# Autodesk Inventor assembly: 足首_独立ピッチ_1
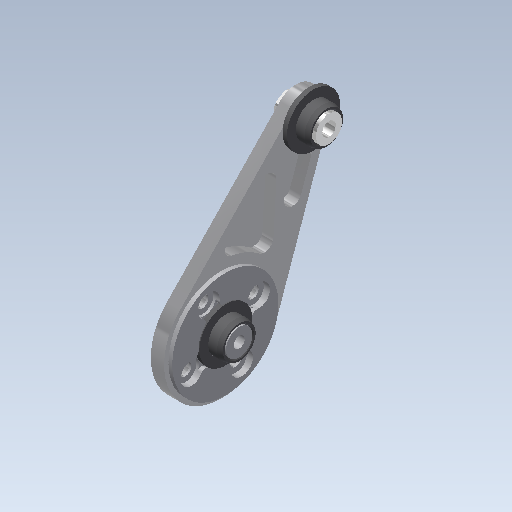
[picture p0: Inventor's stored thumbnail of the model, 512x512]
Saved by Autodesk Inventor 2020 (Build 240168000, 168)
## iProperties
Created: 2016-05-04
Part Number: 足首_独立ピッチ_1
Document SubType Name: Assembly
Designer: hiroaki
Mass: 12.4515 g
Surface Area: 78.9605 cm^2
Volume: 4.53639 cm^3
Density: 2.74481 g/cm^3
Author: hiroaki
## Documents named in this file (6)
- C:\Users\Masato\Desktop\最新版\OpenPlatform_ver3_0\下半身\足首\足首_独立ピッチ_1.iam
- C:\Users\Masato\Desktop\最新版\OpenPlatform_ver3_0\下半身\足首\足首_独立ピッチ_1_1.ipt
- C:\Users\Masato\Desktop\最新版\OpenPlatform_ver3_0\下半身\足首\足首_独立ピッチ_1_2.ipt
- C:\Users\Masato\Desktop\最新版\OpenPlatform_ver3_0\Ready_Made\CU-306.ipt
- C:\Users\Masato\Desktop\最新版\OpenPlatform_ver3_0\Ready_Made\S3-07-3W.ipt
- C:\Users\Masato\Desktop\最新版\OpenPlatform_ver3_0\Ready_Made\80F-0603.ipt
## Components (6 placed, 5 different names)
1. 足首_独立ピッチ_1_1:1 — 挿入:1, 挿入:4, 挿入:5, 挿入:6, 挿入:8
2. 足首_独立ピッチ_1_2:1 — 挿入:1, 挿入:7, 挿入:8
3. CU-306:1 — 挿入:5
4. S3-07-3W:1 — 挿入:4
5. 80F-0603:1 — 挿入:6
6. 80F-0603:2 — 挿入:7
## Relationships (6: Insert 6)
- 挿入:1 [Insert]: 足首_独立ピッチ_1_1:1 ↔ 足首_独立ピッチ_1_2:1
- 挿入:4 [Insert]: 足首_独立ピッチ_1_1:1 ↔ S3-07-3W:1
- 挿入:5 [Insert]: 足首_独立ピッチ_1_1:1 ↔ CU-306:1
- 挿入:6 [Insert]: 足首_独立ピッチ_1_1:1 ↔ 80F-0603:1
- 挿入:7 [Insert]: 足首_独立ピッチ_1_2:1 ↔ 80F-0603:2
- 挿入:8 [Insert]: 足首_独立ピッチ_1_1:1 ↔ 足首_独立ピッチ_1_2:1
